# Autodesk Inventor assembly: Gantry Assembly
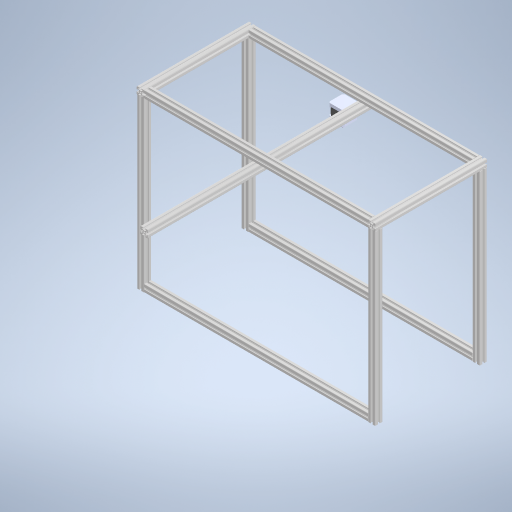
[picture p0: Inventor's stored thumbnail of the model, 512x512]
Saved by Autodesk Inventor 2023 (Build 270158000, 158)
## iProperties
Created: 2023-01-25
Part Number: Gantry Assembly
Document SubType Name: Assembly
Designer: Steven
Author: Steven
## Documents named in this file (12)
- C:\Users\steve\OneDrive\Documents\McMaster University\Courses-Year5\4TB6 Capstone Design Project\The_Nursery_Project\parts\Tray Dropper\Gantry\Gantry Assembly.iam
- C:\Users\steve\Downloads\5537T012_T-Slotted Framing - 1.5ft.ipt
- C:\Users\steve\Downloads\5537T751_T-Slotted Framing - 2ft.ipt
- C:\Users\steve\Downloads\5537T228_T-Slotted Framing - 1ft.ipt
- C:\Users\steve\Downloads\5537T012_T-Slotted Framing - 1.5ft_MIR.ipt
- C:\Users\steve\Downloads\5537T751_T-Slotted Framing - 2ft_MIR.ipt
- C:\Users\steve\Downloads\5537T228_T-Slotted Framing - 1ft_MIR.ipt
- C:\Users\steve\Downloads\5537T012_T-Slotted Framing - 1.5ft_MIR1.ipt
- C:\Users\steve\Downloads\5537T012_T-Slotted Framing - 1.5ft_MIR_MIR.ipt
- C:\Users\steve\Downloads\5537T751_T-Slotted Framing - 2ft_MIR1.ipt
- C:\Users\steve\Downloads\5537T751_T-Slotted Framing - 2ft_MIR_MIR.ipt
- C:\Users\steve\Downloads\nema-17-41.snapshot.2\Nema 17 stepper.ipt
## Components (12 placed, 11 different names)
1. 5537T012_T-Slotted Framing - 1.5ft:1 — Mate:1, Flush:1, Flush:2, Flush:5, Flush:6
2. 5537T751_T-Slotted Framing - 2ft:1 — Mate:2, Flush:3, Flush:4, Flush:9, Mate:5, Mate:6, Mate:8
3. 5537T228_T-Slotted Framing - 1ft:1 — Mate:1, Flush:1, Flush:2, Mate:2, Flush:3, Flush:4
4. 5537T012_T-Slotted Framing - 1.5ft_MIR:1 — Flush:7, Flush:8
5. 5537T751_T-Slotted Framing - 2ft_MIR:1
6. 5537T228_T-Slotted Framing - 1ft_MIR:1
7. 5537T012_T-Slotted Framing - 1.5ft_MIR1:1 — Mate:4
8. 5537T012_T-Slotted Framing - 1.5ft_MIR_MIR:1 — Mate:3
9. 5537T751_T-Slotted Framing - 2ft_MIR1:1 — Flush:5, Flush:6, Mate:4
10. 5537T751_T-Slotted Framing - 2ft_MIR_MIR:1 — Flush:7, Flush:8, Mate:3
11. 5537T751_T-Slotted Framing - 2ft:2 — Flush:9, Mate:5, Mate:6, Mate:7, Flush:10
12. Nema 17 stepper:1 — Mate:7, Mate:8, Flush:10
## Relationships (18: Flush 10, Mate 8)
- Mate:1: 5537T012_T-Slotted Framing - 1.5ft:1 ↔ 5537T228_T-Slotted Framing - 1ft:1
- Flush:1: 5537T012_T-Slotted Framing - 1.5ft:1 ↔ 5537T228_T-Slotted Framing - 1ft:1
- Flush:2: 5537T012_T-Slotted Framing - 1.5ft:1 ↔ 5537T228_T-Slotted Framing - 1ft:1
- Mate:2: 5537T751_T-Slotted Framing - 2ft:1 ↔ 5537T228_T-Slotted Framing - 1ft:1
- Flush:3: 5537T751_T-Slotted Framing - 2ft:1 ↔ 5537T228_T-Slotted Framing - 1ft:1
- Flush:4: 5537T751_T-Slotted Framing - 2ft:1 ↔ 5537T228_T-Slotted Framing - 1ft:1
- Flush:5: 5537T012_T-Slotted Framing - 1.5ft:1 ↔ 5537T751_T-Slotted Framing - 2ft_MIR1:1
- Flush:6: 5537T012_T-Slotted Framing - 1.5ft:1 ↔ 5537T751_T-Slotted Framing - 2ft_MIR1:1
- Flush:7: 5537T012_T-Slotted Framing - 1.5ft_MIR:1 ↔ 5537T751_T-Slotted Framing - 2ft_MIR_MIR:1
- Flush:8: 5537T012_T-Slotted Framing - 1.5ft_MIR:1 ↔ 5537T751_T-Slotted Framing - 2ft_MIR_MIR:1
- Mate:3: 5537T012_T-Slotted Framing - 1.5ft_MIR_MIR:1 ↔ 5537T751_T-Slotted Framing - 2ft_MIR_MIR:1
- Mate:4: 5537T012_T-Slotted Framing - 1.5ft_MIR1:1 ↔ 5537T751_T-Slotted Framing - 2ft_MIR1:1
- Flush:9: 5537T751_T-Slotted Framing - 2ft:1 ↔ 5537T751_T-Slotted Framing - 2ft:2
- Mate:5: 5537T751_T-Slotted Framing - 2ft:1 ↔ 5537T751_T-Slotted Framing - 2ft:2
- Mate:6: 5537T751_T-Slotted Framing - 2ft:1 ↔ 5537T751_T-Slotted Framing - 2ft:2
- Mate:7: 5537T751_T-Slotted Framing - 2ft:2 ↔ Nema 17 stepper:1
- Mate:8 (5.08 mm): 5537T751_T-Slotted Framing - 2ft:1 ↔ Nema 17 stepper:1
- Flush:10 (15.875 mm): 5537T751_T-Slotted Framing - 2ft:2 ↔ Nema 17 stepper:1
